# Autodesk Inventor assembly: ASY PRS 9600 accses hatch
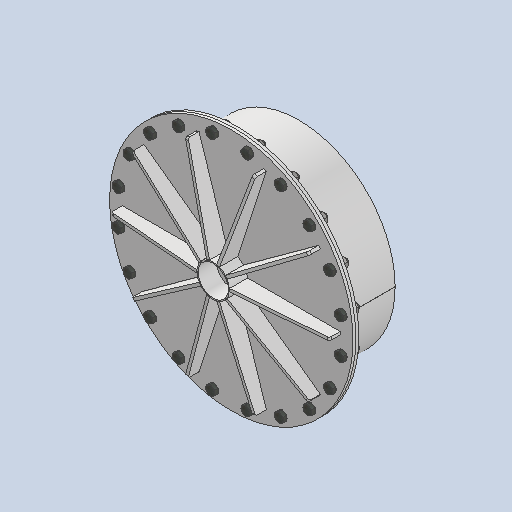
[picture p0: Inventor's stored thumbnail of the model, 512x512]
Saved by Autodesk Inventor 2026.2 (Build 302298000, 298)
## iProperties
Created: 2026-06-21
Part Number: ASY PRS 9600 accses hatch
Document SubType Name: Assembly
Designer: admin
Author: admin
## Documents named in this file (7)
- C:\Users\admin\Documents\Inventor\PRS-Purovsk\ASY PRS 9600 accses hatch.iam
- C:\Users\admin\Documents\Inventor\PRS-Purovsk\ASY PRS 1610 charging hatch_D1200 940.iam
- C:\Users\admin\Documents\Inventor\PRS-Purovsk\PRS 9612 accses hatch flangeipt_D1200 940.ipt
- C:\Users\admin\Documents\Inventor\PRS-Purovsk\PRS 9311 accses hatch tube_D1200 940.ipt
- C:\Users\admin\Documents\Inventor\PRS-Purovsk\cc\en-US\ISO 4018\ISO 4018 - M16 x 40.ipt
- C:\Users\admin\Documents\Inventor\PRS-Purovsk\cc\en-US\ISO 7089\ISO 7089 - 16 - 140 HV(1).ipt
- C:\Users\admin\Documents\Inventor\PRS-Purovsk\cc\en-US\ISO 4032(2)\ISO 4032 - M16 - ISO.ipt
## Components (63 placed, 6 different names)
1. ASY PRS 1610 charging hatch_D1200 940:1 [sub-assembly]
2. PRS 9612 accses hatch flangeipt_D1200 940:1
3. PRS 9311 accses hatch tube_D1200 940:1
4. ISO 4018 M16 x 40:1
5. ISO 7089 16:1
6. ISO 4032 M16:1
7. ISO 4018 M16 x 40:2
8. ISO 4018 M16 x 40:3
9. ISO 4018 M16 x 40:4
10. ISO 4018 M16 x 40:5
11. ISO 4018 M16 x 40:6
12. ISO 4018 M16 x 40:7
13. ISO 4018 M16 x 40:8
14. ISO 4018 M16 x 40:9
15. ISO 4018 M16 x 40:10
16. ISO 4018 M16 x 40:11
17. ISO 4018 M16 x 40:12
18. ISO 4018 M16 x 40:13
19. ISO 4018 M16 x 40:14
20. ISO 4018 M16 x 40:15
21. ISO 4018 M16 x 40:16
22. ISO 4018 M16 x 40:17
23. ISO 4018 M16 x 40:18
24. ISO 4018 M16 x 40:19
25. ISO 4018 M16 x 40:20
26. ISO 7089 16:2
27. ISO 7089 16:3
28. ISO 7089 16:4
29. ISO 7089 16:5
30. ISO 7089 16:6
31. ISO 7089 16:7
32. ISO 7089 16:8
33. ISO 7089 16:9
34. ISO 7089 16:10
35. ISO 7089 16:11
36. ISO 7089 16:12
37. ISO 7089 16:13
38. ISO 7089 16:14
39. ISO 7089 16:15
40. ISO 7089 16:16
41. ISO 7089 16:17
42. ISO 7089 16:18
43. ISO 7089 16:19
44. ISO 7089 16:20
45. ISO 4032 M16:2
46. ISO 4032 M16:3
47. ISO 4032 M16:4
48. ISO 4032 M16:5
49. ISO 4032 M16:6
50. ISO 4032 M16:7
51. ISO 4032 M16:8
52. ISO 4032 M16:9
53. ISO 4032 M16:10
54. ISO 4032 M16:11
55. ISO 4032 M16:12
56. ISO 4032 M16:13
57. ISO 4032 M16:14
58. ISO 4032 M16:15
59. ISO 4032 M16:16
60. ISO 4032 M16:17
61. ISO 4032 M16:18
62. ISO 4032 M16:19
63. ISO 4032 M16:20
## Relationships (102: Mate 80, Insert 20, WeldJoint 2)
- [Mate]: ASY PRS 1610 charging hatch_D1200 940:1 ↔ ISO 4018 M16 x 40:1
- [Mate]: ASY PRS 1610 charging hatch_D1200 940:1 ↔ ISO 4018 M16 x 40:1
- [Mate]: PRS 9612 accses hatch flangeipt_D1200 940:1 ↔ ISO 7089 16:1
- [Mate]: ASY PRS 1610 charging hatch_D1200 940:1 ↔ ISO 7089 16:1
- [Insert]: ISO 7089 16:1 ↔ ISO 4032 M16:1
- [Mate]: ASY PRS 1610 charging hatch_D1200 940:1 ↔ ISO 4018 M16 x 40:2
- [Mate]: ASY PRS 1610 charging hatch_D1200 940:1 ↔ ISO 4018 M16 x 40:2
- [Mate]: ASY PRS 1610 charging hatch_D1200 940:1 ↔ ISO 4018 M16 x 40:3
- [Mate]: ASY PRS 1610 charging hatch_D1200 940:1 ↔ ISO 4018 M16 x 40:3
- [Mate]: ASY PRS 1610 charging hatch_D1200 940:1 ↔ ISO 4018 M16 x 40:4
- [Mate]: ASY PRS 1610 charging hatch_D1200 940:1 ↔ ISO 4018 M16 x 40:4
- [Mate]: ASY PRS 1610 charging hatch_D1200 940:1 ↔ ISO 4018 M16 x 40:5
- [Mate]: ASY PRS 1610 charging hatch_D1200 940:1 ↔ ISO 4018 M16 x 40:5
- [Mate]: ASY PRS 1610 charging hatch_D1200 940:1 ↔ ISO 4018 M16 x 40:6
- [Mate]: ASY PRS 1610 charging hatch_D1200 940:1 ↔ ISO 4018 M16 x 40:6
- [Mate]: ASY PRS 1610 charging hatch_D1200 940:1 ↔ ISO 4018 M16 x 40:7
- [Mate]: ASY PRS 1610 charging hatch_D1200 940:1 ↔ ISO 4018 M16 x 40:7
- [Mate]: ASY PRS 1610 charging hatch_D1200 940:1 ↔ ISO 4018 M16 x 40:8
- [Mate]: ASY PRS 1610 charging hatch_D1200 940:1 ↔ ISO 4018 M16 x 40:8
- [Mate]: ASY PRS 1610 charging hatch_D1200 940:1 ↔ ISO 4018 M16 x 40:9
- [Mate]: ASY PRS 1610 charging hatch_D1200 940:1 ↔ ISO 4018 M16 x 40:9
- [Mate]: ASY PRS 1610 charging hatch_D1200 940:1 ↔ ISO 4018 M16 x 40:10
- [Mate]: ASY PRS 1610 charging hatch_D1200 940:1 ↔ ISO 4018 M16 x 40:10
- [Mate]: ASY PRS 1610 charging hatch_D1200 940:1 ↔ ISO 4018 M16 x 40:11
- [Mate]: ASY PRS 1610 charging hatch_D1200 940:1 ↔ ISO 4018 M16 x 40:11
- [Mate]: ASY PRS 1610 charging hatch_D1200 940:1 ↔ ISO 4018 M16 x 40:12
- [Mate]: ASY PRS 1610 charging hatch_D1200 940:1 ↔ ISO 4018 M16 x 40:12
- [Mate]: ASY PRS 1610 charging hatch_D1200 940:1 ↔ ISO 4018 M16 x 40:13
- [Mate]: ASY PRS 1610 charging hatch_D1200 940:1 ↔ ISO 4018 M16 x 40:13
- [Mate]: ASY PRS 1610 charging hatch_D1200 940:1 ↔ ISO 4018 M16 x 40:14
- [Mate]: ASY PRS 1610 charging hatch_D1200 940:1 ↔ ISO 4018 M16 x 40:14
- [Mate]: ASY PRS 1610 charging hatch_D1200 940:1 ↔ ISO 4018 M16 x 40:15
- [Mate]: ASY PRS 1610 charging hatch_D1200 940:1 ↔ ISO 4018 M16 x 40:15
- [Mate]: ASY PRS 1610 charging hatch_D1200 940:1 ↔ ISO 4018 M16 x 40:16
- [Mate]: ASY PRS 1610 charging hatch_D1200 940:1 ↔ ISO 4018 M16 x 40:16
- [Mate]: ASY PRS 1610 charging hatch_D1200 940:1 ↔ ISO 4018 M16 x 40:17
- [Mate]: ASY PRS 1610 charging hatch_D1200 940:1 ↔ ISO 4018 M16 x 40:17
- [Mate]: ASY PRS 1610 charging hatch_D1200 940:1 ↔ ISO 4018 M16 x 40:18
- [Mate]: ASY PRS 1610 charging hatch_D1200 940:1 ↔ ISO 4018 M16 x 40:18
- [Mate]: ASY PRS 1610 charging hatch_D1200 940:1 ↔ ISO 4018 M16 x 40:19
- [Mate]: ASY PRS 1610 charging hatch_D1200 940:1 ↔ ISO 4018 M16 x 40:19
- [Mate]: ASY PRS 1610 charging hatch_D1200 940:1 ↔ ISO 4018 M16 x 40:20
- [Mate]: ASY PRS 1610 charging hatch_D1200 940:1 ↔ ISO 4018 M16 x 40:20
- [Mate]: PRS 9612 accses hatch flangeipt_D1200 940:1 ↔ ISO 7089 16:2
- [Mate]: ASY PRS 1610 charging hatch_D1200 940:1 ↔ ISO 7089 16:2
- [Mate]: PRS 9612 accses hatch flangeipt_D1200 940:1 ↔ ISO 7089 16:3
- [Mate]: ASY PRS 1610 charging hatch_D1200 940:1 ↔ ISO 7089 16:3
- [Mate]: PRS 9612 accses hatch flangeipt_D1200 940:1 ↔ ISO 7089 16:4
- [Mate]: ASY PRS 1610 charging hatch_D1200 940:1 ↔ ISO 7089 16:4
- [Mate]: PRS 9612 accses hatch flangeipt_D1200 940:1 ↔ ISO 7089 16:5
- [Mate]: ASY PRS 1610 charging hatch_D1200 940:1 ↔ ISO 7089 16:5
- [Mate]: PRS 9612 accses hatch flangeipt_D1200 940:1 ↔ ISO 7089 16:6
- [Mate]: ASY PRS 1610 charging hatch_D1200 940:1 ↔ ISO 7089 16:6
- [Mate]: PRS 9612 accses hatch flangeipt_D1200 940:1 ↔ ISO 7089 16:7
- [Mate]: ASY PRS 1610 charging hatch_D1200 940:1 ↔ ISO 7089 16:7
- [Mate]: PRS 9612 accses hatch flangeipt_D1200 940:1 ↔ ISO 7089 16:8
- [Mate]: ASY PRS 1610 charging hatch_D1200 940:1 ↔ ISO 7089 16:8
- [Mate]: PRS 9612 accses hatch flangeipt_D1200 940:1 ↔ ISO 7089 16:9
- [Mate]: ASY PRS 1610 charging hatch_D1200 940:1 ↔ ISO 7089 16:9
- [Mate]: PRS 9612 accses hatch flangeipt_D1200 940:1 ↔ ISO 7089 16:10
- [Mate]: ASY PRS 1610 charging hatch_D1200 940:1 ↔ ISO 7089 16:10
- [Mate]: PRS 9612 accses hatch flangeipt_D1200 940:1 ↔ ISO 7089 16:11
- [Mate]: ASY PRS 1610 charging hatch_D1200 940:1 ↔ ISO 7089 16:11
- [Mate]: PRS 9612 accses hatch flangeipt_D1200 940:1 ↔ ISO 7089 16:12
- [Mate]: ASY PRS 1610 charging hatch_D1200 940:1 ↔ ISO 7089 16:12
- [Mate]: PRS 9612 accses hatch flangeipt_D1200 940:1 ↔ ISO 7089 16:13
- [Mate]: ASY PRS 1610 charging hatch_D1200 940:1 ↔ ISO 7089 16:13
- [Mate]: PRS 9612 accses hatch flangeipt_D1200 940:1 ↔ ISO 7089 16:14
- [Mate]: ASY PRS 1610 charging hatch_D1200 940:1 ↔ ISO 7089 16:14
- [Mate]: PRS 9612 accses hatch flangeipt_D1200 940:1 ↔ ISO 7089 16:15
- [Mate]: ASY PRS 1610 charging hatch_D1200 940:1 ↔ ISO 7089 16:15
- [Mate]: PRS 9612 accses hatch flangeipt_D1200 940:1 ↔ ISO 7089 16:16
- [Mate]: ASY PRS 1610 charging hatch_D1200 940:1 ↔ ISO 7089 16:16
- [Mate]: PRS 9612 accses hatch flangeipt_D1200 940:1 ↔ ISO 7089 16:17
- [Mate]: ASY PRS 1610 charging hatch_D1200 940:1 ↔ ISO 7089 16:17
- [Mate]: PRS 9612 accses hatch flangeipt_D1200 940:1 ↔ ISO 7089 16:18
- [Mate]: ASY PRS 1610 charging hatch_D1200 940:1 ↔ ISO 7089 16:18
- [Mate]: PRS 9612 accses hatch flangeipt_D1200 940:1 ↔ ISO 7089 16:19
- [Mate]: ASY PRS 1610 charging hatch_D1200 940:1 ↔ ISO 7089 16:19
- [Mate]: PRS 9612 accses hatch flangeipt_D1200 940:1 ↔ ISO 7089 16:20
- [Mate]: ASY PRS 1610 charging hatch_D1200 940:1 ↔ ISO 7089 16:20
- [Insert]: ISO 7089 16:2 ↔ ISO 4032 M16:2
- [Insert]: ISO 7089 16:3 ↔ ISO 4032 M16:3
- [Insert]: ISO 7089 16:4 ↔ ISO 4032 M16:4
- [Insert]: ISO 7089 16:5 ↔ ISO 4032 M16:5
- [Insert]: ISO 7089 16:6 ↔ ISO 4032 M16:6
- [Insert]: ISO 7089 16:7 ↔ ISO 4032 M16:7
- [Insert]: ISO 7089 16:8 ↔ ISO 4032 M16:8
- [Insert]: ISO 7089 16:9 ↔ ISO 4032 M16:9
- [Insert]: ISO 7089 16:10 ↔ ISO 4032 M16:10
- [Insert]: ISO 7089 16:11 ↔ ISO 4032 M16:11
- [Insert]: ISO 7089 16:12 ↔ ISO 4032 M16:12
- [Insert]: ISO 7089 16:13 ↔ ISO 4032 M16:13
- [Insert]: ISO 7089 16:14 ↔ ISO 4032 M16:14
- [Insert]: ISO 7089 16:15 ↔ ISO 4032 M16:15
- [Insert]: ISO 7089 16:16 ↔ ISO 4032 M16:16
- [Insert]: ISO 7089 16:17 ↔ ISO 4032 M16:17
- [Insert]: ISO 7089 16:18 ↔ ISO 4032 M16:18
- [Insert]: ISO 7089 16:19 ↔ ISO 4032 M16:19
- [Insert]: ISO 7089 16:20 ↔ ISO 4032 M16:20
- [WeldJoint]: ASY PRS 1610 charging hatch_D1200 940:1 ↔ PRS 9612 accses hatch flangeipt_D1200 940:1
- [WeldJoint]: PRS 9612 accses hatch flangeipt_D1200 940:1 ↔ PRS 9311 accses hatch tube_D1200 940:1
## Named parameters: d1_d92 = 0 mm, d2_d93 = 0 mm, d3_d94 = 0 mm, d4_d95 = 0 mm, d5_d96 = 0 mm, d6_d97 = 0 mm, d7_d98 = 0 mm, d8_d99 = 0 mm, d9_d100 = 0 mm, d10_d101 = 0 mm, d24_d58 = 0 mm, d25_d59 = 0 mm, d26_d60 = 0 mm, d27_d61 = 0 mm, d28_d62 = 0 mm, d29_d63 = 0 mm, d30_d64 = 0 mm, d31_d65 = 0 mm, d32_d66 = 0 mm, d33_d67 = 0 mm, d34_d68 = 0 mm, d35_d69 = 0 mm, d36_d70 = 0 mm, d37_d71 = 0 mm, d38_d72 = 0 mm, d39_d73 = 0 mm, d40_d74 = 0 mm, d41_d75 = 0 mm, d42_d76 = 0 mm, d43_d77 = 0 mm, d44_d78 = 0 mm, d45_d79 = 0 mm, d46_d80 = 0 mm, d47_d81 = 0 mm, d48_d82 = 0 mm, d49_d83 = 0 mm, d50_d84 = 0 mm, d51_d85 = 0 mm, d52_d86 = 0 mm, d53_d87 = 0 mm, d54_d88 = 0 mm, d55_d89 = 0 mm, d56_d90 = 0 mm, d57_d91 = 0 mm
